# Autodesk Inventor assembly: iDISCO-Sampleholder-Assembly-HumanBrainChunk
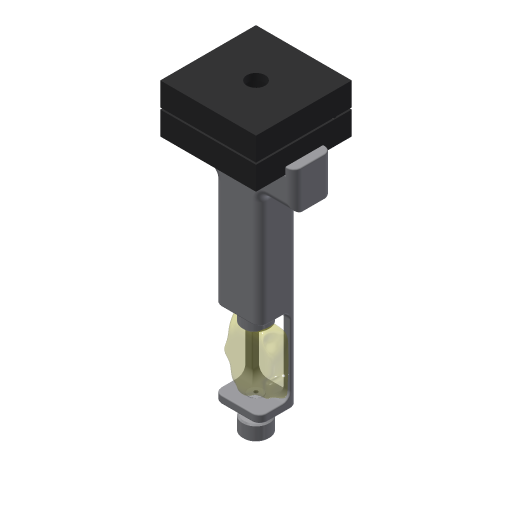
[picture p0: Inventor's stored thumbnail of the model, 512x512]
Saved by Autodesk Inventor 2023 (Build 270158000, 158)
## iProperties
Created: 2019-02-05
Part Number: iDISCO-Sampleholder-Assembly-HumanBrainChunk
Document SubType Name: Assembly
Designer: voigt
Author: voigt
## Documents named in this file (5)
- C:\Users\Public\github\benchtop-hardware\Benchtop\custom-parts\legacy\sample_handling\IDISCO-Sampleholder\iDISCO-Sampleholder-Assembly-HumanBrainChunk.iam
- C:\Users\Public\github\benchtop-hardware\Benchtop\CAD-model-Inventor\library\Thorlabs\kinematic_bases\KB25_M-Step.ipt
- C:\Users\Public\github\benchtop-hardware\Benchtop\custom-parts\legacy\sample_handling\IDISCO-Sampleholder\IDISCO-Sampleholder-12mm-60mm_V2_Sascha.ipt
- C:\Users\Public\github\benchtop-hardware\Benchtop\custom-parts\legacy\sample_handling\IDISCO-Sampleholder\HumanBrainChunk.ipt
- C:\Users\Public\github\benchtop-hardware\Benchtop\CAD-model-Inventor\library\Thorlabs\other\screwM4-12mm.ipt
## Components (5 placed, 4 different names)
1. KB25_M-Step:1 — Insert:1
2. IDISCO-Sampleholder-12mm-60mm_V2_Sascha:1 — Insert:1, Flush:1, Insert:2, Insert:3
3. HumanBrainChunk:1 — Flush:1
4. screwM4-12mm:1 — Insert:3
5. screwM4-12mm:2 — Insert:2
## Relationships (4: Insert 3, Flush 1)
- Insert:1: KB25_M-Step:1 ↔ IDISCO-Sampleholder-12mm-60mm_V2_Sascha:1
- Flush:1 (-5 mm): IDISCO-Sampleholder-12mm-60mm_V2_Sascha:1 ↔ HumanBrainChunk:1
- Insert:2: IDISCO-Sampleholder-12mm-60mm_V2_Sascha:1 ↔ screwM4-12mm:2
- Insert:3 (3 mm): IDISCO-Sampleholder-12mm-60mm_V2_Sascha:1 ↔ screwM4-12mm:1
